# Autodesk Inventor assembly: Odometry module + guards assembly
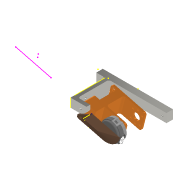
[picture p0: Inventor's stored thumbnail of the model, 180x180]
Saved by Autodesk Inventor 2020 (Build 240168000, 168)
## iProperties
Created: 2020-01-15
Part Number: Odometry module + guards assembly
Document SubType Name: Assembly
Designer: ball
Author: ball
## Documents named in this file (5)
- C:\FTC\FTC8863CAD\2019 Robot\Odoemetry module\Odometry module + guards assembly.iam
- C:\FTC\FTC8863CAD\2019 Robot\Odoemetry module\Odometry_Holder with guard mount.ipt
- C:\FTC\FTC8863CAD\2019 Robot\Odoemetry module\E8T-X-250-S-D-D-X.iam
- C:\FTC\FTC8863CAD\2019 Robot\Odoemetry module\middleMountBracket.ipt
- C:\FTC\FTC8863CAD\2019 Robot\Odoemetry module\encoder guard mirror.ipt
## Components (4 placed, 4 different names)
1. Odometry_Holder with guard mount:1 — Mate:1, Mate:2, Mate:3, Flush:1, Insert:1, Mate:4, Mate:5, Flush:2, Flush:3, Mate:6
2. E8T-X-250-S-D-D-X:1 [sub-assembly] — Mate:1, Mate:2, Mate:3
3. middleMountBracket:1 — Insert:1, Mate:4, Mate:6
4. encoder guard mirror:1 — Mate:5, Flush:2, Flush:3
## Relationships (10: Mate 6, Flush 3, Insert 1)
- Mate:1: Odometry_Holder with guard mount:1 ↔ E8T-X-250-S-D-D-X:1
- Mate:2: Odometry_Holder with guard mount:1 ↔ E8T-X-250-S-D-D-X:1
- Mate:3: Odometry_Holder with guard mount:1 ↔ E8T-X-250-S-D-D-X:1
- Flush:1 (-10.16 mm): Odometry_Holder with guard mount:1
- Insert:1: Odometry_Holder with guard mount:1 ↔ middleMountBracket:1
- Mate:4: Odometry_Holder with guard mount:1 ↔ middleMountBracket:1
- Mate:5: Odometry_Holder with guard mount:1 ↔ encoder guard mirror:1
- Flush:2 (4.699 mm): Odometry_Holder with guard mount:1 ↔ encoder guard mirror:1
- Flush:3 (5.08 mm): Odometry_Holder with guard mount:1 ↔ encoder guard mirror:1
- Mate:6: Odometry_Holder with guard mount:1 ↔ middleMountBracket:1
